# Autodesk Inventor assembly: Chassis
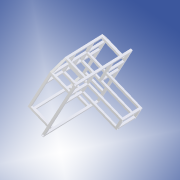
[picture p0: Inventor's stored thumbnail of the model, 180x180]
Saved by Autodesk Inventor 2017 SP1 (Build 210196100, 196)
## iProperties
Created: 2017-06-13
Part Number: Chassis
Document SubType Name: Assembly
Designer: zallen
Mass: 2624.68 g
Surface Area: 12822.9 cm^2
Volume: 1698.76 cm^3
Density: 1.54505 g/cm^3
Author: zallen
## Documents named in this file (11)
- C:\Users\Zach\Documents\GitHub\cr-laundry-robot\src\Base 2\Chassis\Chassis.iam
- C:\Users\Zach\Documents\GitHub\cr-laundry-robot\src\Base 2\Chassis\C001.ipt
- C:\Users\Zach\Documents\GitHub\cr-laundry-robot\src\Base 2\Chassis\C002.ipt
- C:\Users\Zach\Documents\GitHub\cr-laundry-robot\src\Base 2\Chassis\C003.ipt
- C:\Users\Zach\Documents\GitHub\cr-laundry-robot\src\Base 2\Chassis\C006.ipt
- C:\Users\Zach\Documents\GitHub\cr-laundry-robot\src\Base 2\Chassis\C007.ipt
- C:\Users\Zach\Documents\GitHub\cr-laundry-robot\src\Base 2\Chassis\C008.ipt
- C:\Users\Zach\Documents\GitHub\cr-laundry-robot\src\Base 2\Chassis\C010.ipt
- C:\Users\Zach\Documents\GitHub\cr-laundry-robot\src\Base 2\Chassis\C009.ipt
- C:\Users\Zach\Documents\GitHub\cr-laundry-robot\src\Base 2\Chassis\C011.ipt
- C:\Users\Zach\Documents\GitHub\cr-laundry-robot\src\Base 2\Chassis\C012.ipt
## Components (48 placed, 10 different names)
1. C001:1 — Mate:2, Mate:3, Mate:10, Mate:11, Mate:67, Mate:69, Mate:70
2. C001:2 — Mate:4, Mate:5, Mate:12, Mate:13, Mate:64, Mate:65
3. C002:1 — Mate:2, Mate:3, Mate:6, Mate:7
4. C002:2 — Mate:4, Mate:5, Mate:8, Mate:9, Mate:66, Mate:76
5. C003:1 — Mate:6, Mate:7, Mate:8, Mate:9, Mate:75, Mate:77, Mate:78, Mate:135, Mate:143
6. C002:3 — Mate:10, Mate:11, Mate:68, Mate:74
7. C002:4 — Mate:12, Mate:13, Mate:14, Mate:17, Mate:60, Mate:61, Mate:62, Mate:63
8. C003:2 — Mate:14, Mate:17, Mate:60, Mate:61, Mate:62, Mate:71, Mate:72, Mate:73, Mate:130, Mate:165
9. C006:1 — Mate:63, Mate:64
10. C006:2 — Mate:65, Mate:66, Mate:87, Mate:88
11. C006:3 — Mate:67, Mate:68
12. C006:4 — Mate:69, Mate:70, Mate:89, Mate:90
13. C006:5 — Mate:71, Mate:72
14. C006:6 — Mate:73, Mate:74, Mate:94
15. C006:7 — Mate:75, Mate:76, Mate:91
16. C006:8 — Mate:77, Mate:78
17. C007:1 — Mate:87, Mate:88, Mate:92, Mate:96, Flush:19, Flush:21, Mate:179
18. C007:2 — Mate:89, Mate:90, Mate:95
19. C008:1 — Mate:91, Mate:92, Mate:128, Mate:142
20. C008:2 — Mate:94, Mate:95, Mate:96, Mate:125, Mate:167
21. C008:3 — Mate:109, Mate:110, Mate:113, Mate:115, Mate:124, Mate:131, Mate:132, Mate:176, Flush:11, Flush:13, Flush:14, Mate:178, Flush:22, Flush:23, Mate:181, Mate:182
22. C008:4 — Mate:111, Mate:112, Mate:114, Mate:116, Mate:127, Mate:133, Mate:134, Flush:1, Flush:4, Mate:170, Mate:171, Mate:173, Flush:24, Flush:25, Mate:180, Mate:183
23. C010:1 — Mate:109, Mate:110, Mate:111, Mate:112
24. C010:2 — Mate:113, Mate:114, Mate:115, Mate:116, Flush:18, Flush:20, Flush:27, Flush:28, Mate:184, Mate:185
25. C009:1 — Mate:124, Mate:125
26. C009:2 — Mate:127, Mate:128
27. C009:3 — Mate:130, Mate:131, Mate:132
28. C009:4 — Mate:133, Mate:134, Mate:135, Flush:6
29. C009:5 — Mate:142, Mate:144, Flush:5
30. C009:6 — Mate:143, Mate:145, Mate:146
31. C008:5 — Mate:144, Mate:145, Mate:146, Mate:153, Mate:154, Mate:172, Mate:174, Mate:175, Flush:26
32. C010:3 — Mate:153, Mate:154, Mate:155, Mate:156, Mate:163
33. C008:6 — Mate:155, Mate:156, Mate:164, Mate:166, Mate:168, Mate:169, Flush:9, Flush:12, Mate:177
34. C009:7 — Mate:163, Mate:164, Mate:165, Flush:16
35. C009:8 — Mate:166, Mate:167, Flush:17
36. C010:4 — Mate:168, Mate:169, Flush:8, Mate:175, Flush:10
37. C011:1 — Flush:13, Flush:16, Mate:178
38. C011:2 — Flush:14, Mate:177, Flush:17
39. C011:4 — Flush:8, Flush:9, Mate:176, Flush:11, Flush:12
40. C011:5 — Flush:4, Flush:5, Mate:173
41. C011:6 — Flush:1, Mate:170, Mate:171, Mate:172, Flush:10
42. C011:7 — Flush:6, Mate:174, Flush:26
43. C012:1 — Flush:18, Flush:25, Mate:183
44. C012:2 — Flush:19, Flush:24, Mate:179, Mate:180
45. C012:3 — Flush:21, Flush:22, Mate:181
46. C012:4 — Flush:20, Flush:23, Mate:182
47. C011:8 — Flush:27, Mate:184
48. C011:9 — Flush:28, Mate:185
## Relationships (116: Mate 92, Flush 24)
- Mate:2: C001:1 ↔ C002:1
- Mate:3: C001:1 ↔ C002:1
- Mate:4: C001:2 ↔ C002:2
- Mate:5: C001:2 ↔ C002:2
- Mate:6: C002:1 ↔ C003:1
- Mate:7: C002:1 ↔ C003:1
- Mate:8: C002:2 ↔ C003:1
- Mate:9: C002:2 ↔ C003:1
- Mate:10: C001:1 ↔ C002:3
- Mate:11: C001:1 ↔ C002:3
- Mate:12: C001:2 ↔ C002:4
- Mate:13: C001:2 ↔ C002:4
- Mate:14: C002:4 ↔ C003:2
- Mate:17: C002:4 ↔ C003:2
- Mate:60: C002:4 ↔ C003:2
- Mate:61: C002:4 ↔ C003:2
- Mate:62: C002:4 ↔ C003:2
- Mate:63: C002:4 ↔ C006:1
- Mate:64: C001:2 ↔ C006:1
- Mate:65: C001:2 ↔ C006:2
- Mate:66: C002:2 ↔ C006:2
- Mate:67: C001:1 ↔ C006:3
- Mate:68: C002:3 ↔ C006:3
- Mate:69: C001:1 ↔ C006:4
- Mate:70: C001:1 ↔ C006:4
- Mate:71: C003:2 ↔ C006:5
- Mate:72: C003:2 ↔ C006:5
- Mate:73: C003:2 ↔ C006:6
- Mate:74: C002:3 ↔ C006:6
- Mate:75: C003:1 ↔ C006:7
- Mate:76: C002:2 ↔ C006:7
- Mate:77: C003:1 ↔ C006:8
- Mate:78: C003:1 ↔ C006:8
- Mate:87: C006:2 ↔ C007:1
- Mate:88: C006:2 ↔ C007:1
- Mate:89: C006:4 ↔ C007:2
- Mate:90: C006:4 ↔ C007:2
- Mate:91: C006:7 ↔ C008:1
- Mate:92: C007:1 ↔ C008:1
- Mate:94: C006:6 ↔ C008:2
- Mate:95: C007:2 ↔ C008:2
- Mate:96: C007:1 ↔ C008:2
- Mate:109: C008:3 ↔ C010:1
- Mate:110: C008:3 ↔ C010:1
- Mate:111: C008:4 ↔ C010:1
- Mate:112: C008:4 ↔ C010:1
- Mate:113: C008:3 ↔ C010:2
- Mate:114: C008:4 ↔ C010:2
- Mate:115: C008:3 ↔ C010:2
- Mate:116: C008:4 ↔ C010:2
- Mate:124: C008:3 ↔ C009:1
- Mate:125: C008:2 ↔ C009:1
- Mate:127: C008:4 ↔ C009:2
- Mate:128: C008:1 ↔ C009:2
- Mate:130: C003:2 ↔ C009:3
- Mate:131: C008:3 ↔ C009:3
- Mate:132: C008:3 ↔ C009:3
- Mate:133: C008:4 ↔ C009:4
- Mate:134: C008:4 ↔ C009:4
- Mate:135: C003:1 ↔ C009:4
- Mate:142: C008:1 ↔ C009:5
- Mate:143: C003:1 ↔ C009:6
- Mate:144: C009:5 ↔ C008:5
- Mate:145: C009:6 ↔ C008:5
- Mate:146: C009:6 ↔ C008:5
- Mate:153: C008:5 ↔ C010:3
- Mate:154: C008:5 ↔ C010:3
- Mate:155: C010:3 ↔ C008:6
- Mate:156: C010:3 ↔ C008:6
- Mate:163: C010:3 ↔ C009:7
- Mate:164: C008:6 ↔ C009:7
- Mate:165: C003:2 ↔ C009:7
- Mate:166: C008:6 ↔ C009:8
- Mate:167: C008:2 ↔ C009:8
- Mate:168: C008:6 ↔ C010:4
- Mate:169: C008:6 ↔ C010:4
- Flush:1: C008:4 ↔ C011:6
- Flush:4: C008:4 ↔ C011:5
- Flush:5: C009:5 ↔ C011:5
- Mate:170: C008:4 ↔ C011:6
- Mate:171: C008:4 ↔ C011:6
- Mate:172: C008:5 ↔ C011:6
- Mate:173: C008:4 ↔ C011:5
- Flush:6: C009:4 ↔ C011:7
- Mate:174: C008:5 ↔ C011:7
- Flush:8: C010:4 ↔ C011:4
- Flush:9: C008:6 ↔ C011:4
- Mate:175: C008:5 ↔ C010:4
- Flush:10: C010:4 ↔ C011:6
- Mate:176: C008:3 ↔ C011:4
- Flush:11: C008:3 ↔ C011:4
- Flush:12: C008:6 ↔ C011:4
- Flush:13: C008:3 ↔ C011:1
- Flush:14: C008:3 ↔ C011:2
- Mate:177: C008:6 ↔ C011:2
- Flush:16: C009:7 ↔ C011:1
- Mate:178: C008:3 ↔ C011:1
- Flush:17: C009:8 ↔ C011:2
- Flush:18: C010:2 ↔ C012:1
- Flush:19: C007:1 ↔ C012:2
- Flush:20: C010:2 ↔ C012:4
- Flush:21: C007:1 ↔ C012:3
- Flush:22: C008:3 ↔ C012:3
- Flush:23: C008:3 ↔ C012:4
- Flush:24: C008:4 ↔ C012:2
- Flush:25: C008:4 ↔ C012:1
- Mate:179: C007:1 ↔ C012:2
- Mate:180: C008:4 ↔ C012:2
- Mate:181: C008:3 ↔ C012:3
- Mate:182: C008:3 ↔ C012:4
- Mate:183: C008:4 ↔ C012:1
- Flush:26: C008:5 ↔ C011:7
- Flush:27: C010:2 ↔ C011:8
- Flush:28: C010:2 ↔ C011:9
- Mate:184: C010:2 ↔ C011:8
- Mate:185: C010:2 ↔ C011:9
